# Autodesk Inventor assembly: Slider_crank_mechanism
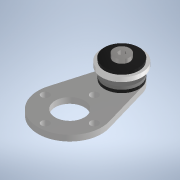
[picture p0: Inventor's stored thumbnail of the model, 180x180]
Saved by Autodesk Inventor 2020.4 (Build 244396000, 396)
## iProperties
Created: 2021-09-06
Part Number: Slider_crank_mechanism
Document SubType Name: Assembly
Designer: Masato Kubotera
Mass: 2.53036 g
Surface Area: 18.5815 cm^2
Volume: 1.13409 cm^3
Density: 2.23118 g/cm^3
Author: Masato Kubotera
## Documents named in this file (8)
- C:\Users\Masato\Documents\Inventor\CIT Brains_Inventor\OpenPlatform_ver3_0（ワッシャ変更）\LowerBody\Slider_crank\Slider_crank_mechanism.iam
- C:\Users\Masato\Documents\Inventor\CIT Brains_Inventor\OpenPlatform_ver3_0（ワッシャ変更）\LowerBody\Slider_crank\Slider_crank_horn.ipt
- C:\Users\Masato\Documents\Inventor\CIT Brains_Inventor\OpenPlatform_ver3_0（ワッシャ変更）\Ready_Made\80F-0603.ipt
- C:\Users\Masato\Documents\Inventor\CIT Brains_Inventor\OpenPlatform_ver3_0（ワッシャ変更）\Ready_Made\UUW-0312-10BH.ipt
- C:\Users\Masato\Documents\Inventor\CIT Brains_Inventor\OpenPlatform_ver3_0（ワッシャ変更）\Ready_Made\ARU-304_5S.ipt
- C:\Users\Masato\Documents\Inventor\CIT Brains_Inventor\OpenPlatform_ver3_0（ワッシャ変更）\Ready_Made\Screw\M3-10.ipt
- C:\Users\Masato\Documents\Inventor\CIT Brains_Inventor\OpenPlatform_ver3_0（ワッシャ変更）\Ready_Made\TT-0814-15.ipt
- C:\Users\Masato\Documents\Inventor\CIT Brains_Inventor\OpenPlatform_ver3_0（ワッシャ変更）\Ready_Made\SF319.ipt
## Components (8 placed, 7 different names)
1. Slider_crank_horn:1 — 挿入:1, 挿入:9
2. 80F-0603:1 — 挿入:2
3. UUW-0312-10BH:1 — 挿入:1, 挿入:2, 挿入:4
4. ARU-304_5S:1 — 挿入:4, 挿入:10
5. UUW-0312-10BH:2 — 挿入:7, 挿入:8, 挿入:10
6. M3-10:1 — 挿入:7
7. TT-0814-15:1 — 挿入:8
8. SF319:1 — 挿入:9
## Relationships (7: Insert 7)
- 挿入:1 [Insert]: Slider_crank_horn:1 ↔ UUW-0312-10BH:1
- 挿入:2 [Insert]: 80F-0603:1 ↔ UUW-0312-10BH:1
- 挿入:4 [Insert]: UUW-0312-10BH:1 ↔ ARU-304_5S:1
- 挿入:7 [Insert]: UUW-0312-10BH:2 ↔ M3-10:1
- 挿入:8 [Insert]: UUW-0312-10BH:2 ↔ TT-0814-15:1
- 挿入:9 [Insert]: Slider_crank_horn:1 ↔ SF319:1
- 挿入:10 [Insert]: ARU-304_5S:1 ↔ UUW-0312-10BH:2
